# Autodesk Inventor assembly: nhk35
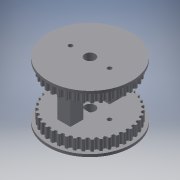
[picture p0: Inventor's stored thumbnail of the model, 180x180]
Saved by Autodesk Inventor 2019 (Build 230136000, 136)
## iProperties
Created: 2022-02-27
Part Number: nhk35
Material: 一般
Document SubType Name: Assembly
Designer: yuta
Author: yuta
## Documents named in this file (4)
- C:\Users\yuta\Documents\NHK\nhk35.iam
- C:\Users\yuta\Documents\NHK\nhk27.ipt
- C:\Users\yuta\Documents\NHK\nhk33.ipt
- C:\Users\yuta\Documents\NHK\nhk34.ipt
## Components (6 placed, 3 different names)
1. nhk27:1 — フラッシュ:1, メイト:1, フラッシュ:2, メイト:2, メイト:3, メイト:4, メイト:12, メイト:13, メイト:14
2. nhk27:2 — フラッシュ:3, メイト:5, メイト:6, メイト:7, メイト:8, メイト:9, メイト:10, メイト:11
3. nhk33:1 — フラッシュ:2, メイト:2, メイト:3, メイト:7, メイト:8
4. nhk33:2 — フラッシュ:1, メイト:1, メイト:4, フラッシュ:3, メイト:5, メイト:6
5. nhk34:1 — メイト:9, メイト:10, メイト:11
6. nhk34:2 — メイト:12, メイト:13, メイト:14
## Relationships (17: Mate 14, Flush 3)
- フラッシュ:1 [Flush]: nhk27:1 ↔ nhk33:2
- メイト:1 [Mate]: nhk27:1 ↔ nhk33:2
- フラッシュ:2 [Flush]: nhk27:1 ↔ nhk33:1
- メイト:2 [Mate]: nhk27:1 ↔ nhk33:1
- メイト:3 [Mate]: nhk27:1 ↔ nhk33:1
- メイト:4 [Mate]: nhk27:1 ↔ nhk33:2
- フラッシュ:3 [Flush]: nhk27:2 ↔ nhk33:2
- メイト:5 [Mate]: nhk27:2 ↔ nhk33:2
- メイト:6 [Mate]: nhk27:2 ↔ nhk33:2
- メイト:7 [Mate]: nhk27:2 ↔ nhk33:1
- メイト:8 [Mate]: nhk27:2 ↔ nhk33:1
- メイト:9 [Mate]: nhk27:2 ↔ nhk34:1
- メイト:10 [Mate]: nhk27:2 ↔ nhk34:1
- メイト:11 [Mate]: nhk27:2 ↔ nhk34:1
- メイト:12 [Mate]: nhk27:1 ↔ nhk34:2
- メイト:13 [Mate]: nhk27:1 ↔ nhk34:2
- メイト:14 [Mate]: nhk27:1 ↔ nhk34:2
